# Autodesk Inventor assembly: 72156
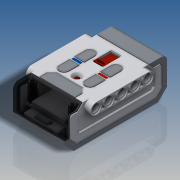
[picture p0: Inventor's stored thumbnail of the model, 180x180]
Saved by Autodesk Inventor 2016 SP2 (Build 200236200, 236)
## iProperties
Created: 2015-08-26
Part Number: 72156
Document SubType Name: Assembly
Designer: D. Kohfeld
Mass: 17.8503 g
Surface Area: 280.533 cm^2
Volume: 15.6075 cm^3
Density: 1.1437 g/cm^3
Author: D. Kohfeld
## Documents named in this file (5)
- A:\LEGO Pieces\EV3\72156.iam
- A:\LEGO Pieces\EV3\76607c01.iam
- A:\LEGO Pieces\EV3\11237-Red.ipt
- A:\LEGO Pieces\EV3\u9013-Black.ipt
- A:\LEGO Pieces\EV3\76609-LtBluishGray.ipt
## Components (4 placed, 4 different names)
1. 76607c01:1 [sub-assembly] — Flush:1, Mate:1, Flush:2, Flush:3, Mate:2, Mate:3
2. 11237-Red:1 — Flush:3, Mate:2, Mate:3
3. u9013-Black:1 — Insert:1
4. 76609-LtBluishGray:1 — Flush:1, Mate:1, Flush:2, Insert:1
## Relationships (7: Flush 3, Mate 3, Insert 1)
- Flush:1: 76607c01:1 ↔ 76609-LtBluishGray:1
- Mate:1: 76607c01:1 ↔ 76609-LtBluishGray:1
- Flush:2: 76607c01:1 ↔ 76609-LtBluishGray:1
- Insert:1: u9013-Black:1 ↔ 76609-LtBluishGray:1
- Flush:3: 76607c01:1 ↔ 11237-Red:1
- Mate:2: 76607c01:1 ↔ 11237-Red:1
- Mate:3: 76607c01:1 ↔ 11237-Red:1
